# Autodesk Inventor assembly: Assembly1_for_rendering
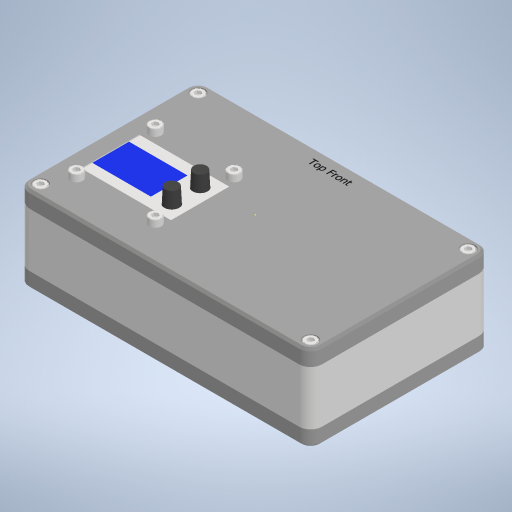
[picture p0: Inventor's stored thumbnail of the model, 512x512]
Saved by Autodesk Inventor 2023 (Build 270158000, 158)
## iProperties
Created: 2023-05-16
Part Number: Assembly1_for_rendering
Document SubType Name: Assembly
Designer: mark
Author: mark
## Documents named in this file (8)
- D:\Egyetem\BME MSc\Diplomamunka\opendaq\cad\assembly\Assembly1_for_rendering.iam
- D:\Egyetem\BME MSc\Diplomamunka\opendaq\cad\housing\housing_bottom.ipt
- D:\Egyetem\BME MSc\Diplomamunka\opendaq\cad\housing\housing_side.ipt
- D:\Egyetem\BME MSc\Diplomamunka\opendaq\cad\housing\housing_top.ipt
- D:\Egyetem\BME MSc\Diplomamunka\opendaq\cad\pcb\pcb_main_populated.ipt
- D:\Egyetem\BME MSc\Diplomamunka\opendaq\cad\misc\screws\din912\din_912-m3x0_5-10-8_8.ipt
- D:\Egyetem\BME MSc\Diplomamunka\opendaq\cad\pcb\display_buttons.ipt
- D:\Egyetem\BME MSc\Diplomamunka\opendaq\cad\housing\dust_cover.ipt
## Components (18 placed, 7 different names)
1. housing_bottom:1 — Mate:1, Mate:2, Mate:3, Mate:4, Flush:1, Flush:2, Mate:14, Mate:15, Mate:16, Mate:17, Mate:18, Mate:19, Mate:20, Mate:21
2. housing_side:1 — Mate:4, Flush:1, Flush:2, Mate:5, Flush:3, Flush:4
3. housing_top:1 — Mate:5, Flush:3, Flush:4, Mate:6, Mate:7, Mate:8, Mate:9, Mate:10, Mate:11, Mate:12, Mate:13, Mate:22, Mate:23, Flush:5, Mate:24, Mate:25, Mate:26, Mate:27, Mate:28, Mate:29, Mate:30, Mate:31
4. pcb_main_populated:1 — Mate:1, Mate:2, Mate:3
5. din_912-m3x0_5-10-8_8:1 — Mate:9, Mate:12
6. din_912-m3x0_5-10-8_8:2 — Mate:7, Mate:8
7. din_912-m3x0_5-10-8_8:3 — Mate:10, Mate:11
8. din_912-m3x0_5-10-8_8:4 — Mate:6, Mate:13
9. din_912-m3x0_5-10-8_8:5 — Mate:18, Mate:21
10. din_912-m3x0_5-10-8_8:6 — Mate:17, Mate:20
11. din_912-m3x0_5-10-8_8:7 — Mate:16, Mate:19
12. din_912-m3x0_5-10-8_8:8 — Mate:14, Mate:15
13. display_buttons:1 — Mate:22, Mate:23, Flush:5, Mate:32, Mate:33, Flush:6
14. din_912-m3x0_5-10-8_8:9 — Mate:24, Mate:25
15. din_912-m3x0_5-10-8_8:10 — Mate:30, Mate:31
16. din_912-m3x0_5-10-8_8:11 — Mate:28, Mate:29
17. din_912-m3x0_5-10-8_8:12 — Mate:26, Mate:27
18. dust_cover:1 — Mate:32, Mate:33, Flush:6
## Relationships (39: Mate 33, Flush 6)
- Mate:1: housing_bottom:1 ↔ pcb_main_populated:1
- Mate:2: housing_bottom:1 ↔ pcb_main_populated:1
- Mate:3: housing_bottom:1 ↔ pcb_main_populated:1
- Mate:4: housing_bottom:1 ↔ housing_side:1
- Flush:1: housing_bottom:1 ↔ housing_side:1
- Flush:2: housing_bottom:1 ↔ housing_side:1
- Mate:5: housing_side:1 ↔ housing_top:1
- Flush:3: housing_side:1 ↔ housing_top:1
- Flush:4: housing_side:1 ↔ housing_top:1
- Mate:6: housing_top:1 ↔ din_912-m3x0_5-10-8_8:4
- Mate:7: housing_top:1 ↔ din_912-m3x0_5-10-8_8:2
- Mate:8: housing_top:1 ↔ din_912-m3x0_5-10-8_8:2
- Mate:9: housing_top:1 ↔ din_912-m3x0_5-10-8_8:1
- Mate:10: housing_top:1 ↔ din_912-m3x0_5-10-8_8:3
- Mate:11: housing_top:1 ↔ din_912-m3x0_5-10-8_8:3
- Mate:12: housing_top:1 ↔ din_912-m3x0_5-10-8_8:1
- Mate:13: housing_top:1 ↔ din_912-m3x0_5-10-8_8:4
- Mate:14: housing_bottom:1 ↔ din_912-m3x0_5-10-8_8:8
- Mate:15: housing_bottom:1 ↔ din_912-m3x0_5-10-8_8:8
- Mate:16: housing_bottom:1 ↔ din_912-m3x0_5-10-8_8:7
- Mate:17: housing_bottom:1 ↔ din_912-m3x0_5-10-8_8:6
- Mate:18: housing_bottom:1 ↔ din_912-m3x0_5-10-8_8:5
- Mate:19: housing_bottom:1 ↔ din_912-m3x0_5-10-8_8:7
- Mate:20: housing_bottom:1 ↔ din_912-m3x0_5-10-8_8:6
- Mate:21: housing_bottom:1 ↔ din_912-m3x0_5-10-8_8:5
- Mate:22: housing_top:1 ↔ display_buttons:1
- Mate:23: housing_top:1 ↔ display_buttons:1
- Flush:5 (0.1 mm): housing_top:1 ↔ display_buttons:1
- Mate:24: housing_top:1 ↔ din_912-m3x0_5-10-8_8:9
- Mate:25: housing_top:1 ↔ din_912-m3x0_5-10-8_8:9
- Mate:26: housing_top:1 ↔ din_912-m3x0_5-10-8_8:12
- Mate:27: housing_top:1 ↔ din_912-m3x0_5-10-8_8:12
- Mate:28: housing_top:1 ↔ din_912-m3x0_5-10-8_8:11
- Mate:29: housing_top:1 ↔ din_912-m3x0_5-10-8_8:11
- Mate:30: housing_top:1 ↔ din_912-m3x0_5-10-8_8:10
- Mate:31: housing_top:1 ↔ din_912-m3x0_5-10-8_8:10
- Mate:32: display_buttons:1 ↔ dust_cover:1
- Mate:33: display_buttons:1 ↔ dust_cover:1
- Flush:6: display_buttons:1 ↔ dust_cover:1
